# Autodesk Inventor assembly: main_frame
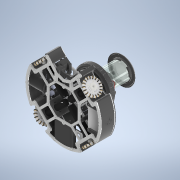
[picture p0: Inventor's stored thumbnail of the model, 180x180]
Saved by Autodesk Inventor 2020 (Build 240168000, 168)
## iProperties
Created: 2024-04-30
Part Number: main_frame
Document SubType Name: Assembly
Designer: 4s
Author: 4s
## Documents named in this file (25)
- C:\Users\4s\Documents\Inventor models\Asterisk\robot_v2\main_frame.iam
- C:\Users\4s\Documents\Inventor models\Asterisk\robot_v2\bottom_plate_v2.ipt
- C:\Users\4s\Documents\Inventor models\Asterisk\robot_v2\maxon mounts\back_mount.ipt
- C:\Users\4s\Documents\Inventor models\Asterisk\robot_v2\maxon mounts\left_mount.ipt
- C:\Users\4s\Documents\Inventor models\Asterisk\robot_v2\maxon mounts\right_mount.ipt
- C:\Users\4s\Documents\Inventor models\Asterisk\robot_v2\maxon motor\maxon motor.iam
- C:\Users\4s\Documents\Inventor models\Asterisk\robot_v2\maxon mounts\inner_mount.ipt
- C:\Users\4s\Documents\Inventor models\Asterisk\robot_v2\side_prot_cap.ipt
- C:\Users\4s\Documents\Inventor models\Asterisk\robot_v2\side_prot_stab_60.ipt
- C:\Users\4s\Documents\Inventor models\Asterisk\robot_v2\Bat_mount\bat_bed003_clear.ipt
- C:\Users\4s\Documents\Inventor models\Asterisk\robot_v2\a1401220.ipt
- C:\Users\4s\Documents\Inventor models\Asterisk\robot_v2\kicker\kicker_base_v7.ipt
- C:\Users\4s\Documents\Inventor models\Asterisk\robot_v2\upper_plate_v2.ipt
- C:\Users\4s\Documents\Inventor models\Asterisk\robot_v2\GTF Robots 50mm Wheel.ipt
- C:\Users\4s\Documents\Inventor models\Asterisk\robot_v2\board_support.ipt
- C:\Users\4s\Documents\Inventor models\Asterisk\robot_v2\pcb_main_board\motherboard.ipt
- C:\Users\4s\Documents\Inventor models\Asterisk\robot_v2\upper_mount\tsop_mount_v5.ipt
- C:\Users\4s\Documents\Inventor models\Asterisk\robot_v2\pcb_tsop_board\asterisk_tsop_board.ipt
- C:\Users\4s\Documents\Inventor models\Asterisk\robot_v2\upper_mount\tsop_imu_v1.ipt
- C:\Users\4s\Documents\Inventor models\Asterisk\9Dof Razor IMU.ipt
- C:\Users\4s\Documents\Inventor models\Asterisk\robot_v2\upper_mount\optic_mount_v3.ipt
- C:\Users\4s\Documents\Inventor models\Asterisk\robot_v2\openmv\openmv_h7.ipt
- C:\Users\4s\Documents\Inventor models\Asterisk\robot_v2\tube_50.ipt
- C:\Users\4s\Documents\Inventor models\Asterisk\robot_v2\mirror_50.ipt
- C:\Users\4s\Documents\Inventor models\Asterisk\robot_v2\upper_mount\mirror_lock_v4.ipt
## Components (34 placed, 24 different names)
1. bottom_plate_v2:1 — Совмещение:1, Совмещение:2, Совмещение:3, Совмещение:4, Совмещение:5, Совмещение:6, Совмещение:7, Совмещение:8, Совмещение:9, Совмещение:10, Совмещение:11, Совмещение:12, Совмещение:22, Совмещение:24, Совмещение:26, Совмещение:28, Совмещение:41, Совмещение:42, Совмещение:43, Совмещение:44, Совмещение:45, Совмещение:46, Совмещение:47, Совмещение:48, Совмещение:49, Совмещение:52, Совмещение:53, Совмещение:54, Совмещение:55
2. back_mount:1 — Совмещение:7, Совмещение:8, Совмещение:9, Совмещение:32, Совмещение:34, Совмещение:58
3. back_mount:2 — Совмещение:10, Совмещение:11, Совмещение:12, Совмещение:29, Совмещение:33, Совмещение:60
4. left_mount:1 — Совмещение:4, Совмещение:5, Совмещение:6, Совмещение:31, Совмещение:35, Совмещение:64
5. right_mount:1 — Совмещение:1, Совмещение:2, Совмещение:3, Совмещение:30, Совмещение:36, Совмещение:62
6. inner_mount:1 — Совмещение:22, Совмещение:38
7. inner_mount:2 — Совмещение:24, Совмещение:39
8. inner_mount:3 — Совмещение:26, Совмещение:40
9. inner_mount:4 — Совмещение:28, Совмещение:37
10. maxon motor:1 [sub-assembly] — Совмещение:30, Совмещение:36, Совмещение:38, Совмещение:61
11. maxon motor:2 [sub-assembly] — Совмещение:31, Совмещение:35, Совмещение:39, Совмещение:63
12. maxon motor:3 [sub-assembly] — Совмещение:32, Совмещение:34, Совмещение:40, Совмещение:57
13. maxon motor:4 [sub-assembly] — Совмещение:29, Совмещение:33, Совмещение:37, Совмещение:59
14. side_prot_cap:1 — Совмещение:41, Совмещение:42, Совмещение:43
15. side_prot_stab_60:1 — Совмещение:44, Совмещение:45, Совмещение:46, Совмещение:50, Совмещение:51
16. bat_bed003_clear:1 — Совмещение:47, Совмещение:48, Совмещение:49
17. a1401220:1 — Совмещение:50, Угол:1, Совмещение:51
18. kicker_base_v7:1 — Совмещение:52, Совмещение:53, Совмещение:54
19. upper_plate_v2:1 — Совмещение:55, Совмещение:56, Заподлицо:1, Совмещение:65, Совмещение:66, Совмещение:67, Совмещение:71, Совмещение:72, Совмещение:73
20. GTF Robots 50mm Wheel:1 — Совмещение:57, Совмещение:58
21. GTF Robots 50mm Wheel:2 — Совмещение:59, Совмещение:60
22. GTF Robots 50mm Wheel:3 — Совмещение:61, Совмещение:62
23. GTF Robots 50mm Wheel:4 — Совмещение:63, Совмещение:64
24. board_support:1 — Совмещение:65, Совмещение:66, Совмещение:67, Совмещение:68, Совмещение:69, Совмещение:70
25. motherboard:1 — Совмещение:68, Совмещение:69, Совмещение:70
26. tsop_mount_v5:1 — Совмещение:71, Совмещение:72, Совмещение:73, Совмещение:74, Совмещение:75, Совмещение:76, Совмещение:77
27. asterisk_tsop_board:1 — Совмещение:74, Совмещение:75, Угол:2, Угол:3
28. tsop_imu_v1:1 — Совмещение:76, Совмещение:77, Совмещение:79, Совмещение:80, Совмещение:81, Угол:5, Совмещение:82
29. 9Dof Razor IMU:1 — Совмещение:78, Совмещение:79, Угол:4
30. optic_mount_v3:1 — Совмещение:80, Совмещение:81, Совмещение:82, Совмещение:83, Совмещение:84, Угол:6, Совмещение:85, Совмещение:86
31. openmv_h7:1 — Совмещение:83, Совмещение:84, Угол:6
32. tube_50:1 — Совмещение:85, Совмещение:86, Совмещение:87, Совмещение:88, Совмещение:89, Угол:7
33. mirror_50:1 — Совмещение:87, Совмещение:88, Совмещение:90
34. mirror_lock_v4:1 — Совмещение:89, Совмещение:90
## Relationships (86: Mate 78, Angle 7, Flush 1)
- Совмещение:1 [Mate]: bottom_plate_v2:1 ↔ right_mount:1
- Совмещение:2 [Mate]: bottom_plate_v2:1 ↔ right_mount:1
- Совмещение:3 [Mate]: bottom_plate_v2:1 ↔ right_mount:1
- Совмещение:4 [Mate]: bottom_plate_v2:1 ↔ left_mount:1
- Совмещение:5 [Mate]: bottom_plate_v2:1 ↔ left_mount:1
- Совмещение:6 [Mate]: bottom_plate_v2:1 ↔ left_mount:1
- Совмещение:7 [Mate]: bottom_plate_v2:1 ↔ back_mount:1
- Совмещение:8 [Mate]: bottom_plate_v2:1 ↔ back_mount:1
- Совмещение:9 [Mate]: bottom_plate_v2:1 ↔ back_mount:1
- Совмещение:10 [Mate]: bottom_plate_v2:1 ↔ back_mount:2
- Совмещение:11 [Mate]: bottom_plate_v2:1 ↔ back_mount:2
- Совмещение:12 [Mate]: bottom_plate_v2:1 ↔ back_mount:2
- Совмещение:22 [Mate]: bottom_plate_v2:1 ↔ inner_mount:1
- Совмещение:24 [Mate]: bottom_plate_v2:1 ↔ inner_mount:2
- Совмещение:26 [Mate]: bottom_plate_v2:1 ↔ inner_mount:3
- Совмещение:28 [Mate]: bottom_plate_v2:1 ↔ inner_mount:4
- Совмещение:29 [Mate]: back_mount:2 ↔ maxon motor:4
- Совмещение:30 [Mate]: right_mount:1 ↔ maxon motor:1
- Совмещение:31 [Mate]: left_mount:1 ↔ maxon motor:2
- Совмещение:32 [Mate]: back_mount:1 ↔ maxon motor:3
- Совмещение:33 [Mate]: back_mount:2 ↔ maxon motor:4
- Совмещение:34 [Mate]: back_mount:1 ↔ maxon motor:3
- Совмещение:35 [Mate]: left_mount:1 ↔ maxon motor:2
- Совмещение:36 [Mate]: right_mount:1 ↔ maxon motor:1
- Совмещение:37 [Mate]: inner_mount:4 ↔ maxon motor:4
- Совмещение:38 [Mate]: inner_mount:1 ↔ maxon motor:1
- Совмещение:39 [Mate]: inner_mount:2 ↔ maxon motor:2
- Совмещение:40 [Mate]: inner_mount:3 ↔ maxon motor:3
- Совмещение:41 [Mate]: bottom_plate_v2:1 ↔ side_prot_cap:1
- Совмещение:42 [Mate]: bottom_plate_v2:1 ↔ side_prot_cap:1
- Совмещение:43 [Mate]: bottom_plate_v2:1 ↔ side_prot_cap:1
- Совмещение:44 [Mate]: bottom_plate_v2:1 ↔ side_prot_stab_60:1
- Совмещение:45 [Mate]: bottom_plate_v2:1 ↔ side_prot_stab_60:1
- Совмещение:46 [Mate]: bottom_plate_v2:1 ↔ side_prot_stab_60:1
- Совмещение:47 [Mate]: bottom_plate_v2:1 ↔ bat_bed003_clear:1
- Совмещение:48 [Mate]: bottom_plate_v2:1 ↔ bat_bed003_clear:1
- Совмещение:49 [Mate]: bottom_plate_v2:1 ↔ bat_bed003_clear:1
- Совмещение:50 [Mate]: side_prot_stab_60:1 ↔ a1401220:1
- Угол:1 [Angle] (0 deg): a1401220:1
- Совмещение:51 [Mate]: side_prot_stab_60:1 ↔ a1401220:1
- Совмещение:52 [Mate]: bottom_plate_v2:1 ↔ kicker_base_v7:1
- Совмещение:53 [Mate]: bottom_plate_v2:1 ↔ kicker_base_v7:1
- Совмещение:54 [Mate]: bottom_plate_v2:1 ↔ kicker_base_v7:1
- Совмещение:55 [Mate] (35 mm): bottom_plate_v2:1 ↔ upper_plate_v2:1
- Совмещение:56 [Mate]: upper_plate_v2:1
- Заподлицо:1 [Flush]: upper_plate_v2:1
- Совмещение:57 [Mate]: maxon motor:3 ↔ GTF Robots 50mm Wheel:1
- Совмещение:58 [Mate] (1.5 mm): back_mount:1 ↔ GTF Robots 50mm Wheel:1
- Совмещение:59 [Mate]: maxon motor:4 ↔ GTF Robots 50mm Wheel:2
- Совмещение:60 [Mate] (1.5 mm): back_mount:2 ↔ GTF Robots 50mm Wheel:2
- Совмещение:61 [Mate]: maxon motor:1 ↔ GTF Robots 50mm Wheel:3
- Совмещение:62 [Mate] (1.5 mm): right_mount:1 ↔ GTF Robots 50mm Wheel:3
- Совмещение:63 [Mate]: maxon motor:2 ↔ GTF Robots 50mm Wheel:4
- Совмещение:64 [Mate] (1.5 mm): left_mount:1 ↔ GTF Robots 50mm Wheel:4
- Совмещение:65 [Mate]: upper_plate_v2:1 ↔ board_support:1
- Совмещение:66 [Mate]: upper_plate_v2:1 ↔ board_support:1
- Совмещение:67 [Mate]: upper_plate_v2:1 ↔ board_support:1
- Совмещение:68 [Mate]: board_support:1 ↔ motherboard:1
- Совмещение:69 [Mate]: board_support:1 ↔ motherboard:1
- Совмещение:70 [Mate]: board_support:1 ↔ motherboard:1
- Совмещение:71 [Mate]: upper_plate_v2:1 ↔ tsop_mount_v5:1
- Совмещение:72 [Mate]: upper_plate_v2:1 ↔ tsop_mount_v5:1
- Совмещение:73 [Mate]: upper_plate_v2:1 ↔ tsop_mount_v5:1
- Совмещение:74 [Mate]: tsop_mount_v5:1 ↔ asterisk_tsop_board:1
- Совмещение:75 [Mate]: tsop_mount_v5:1 ↔ asterisk_tsop_board:1
- Угол:2 [Angle] (0 deg): asterisk_tsop_board:1
- Совмещение:76 [Mate]: tsop_mount_v5:1 ↔ tsop_imu_v1:1
- Совмещение:77 [Mate]: tsop_mount_v5:1 ↔ tsop_imu_v1:1
- Угол:3 [Angle] (0 deg): asterisk_tsop_board:1
- Совмещение:78 [Mate]: 9Dof Razor IMU:1
- Совмещение:79 [Mate]: tsop_imu_v1:1 ↔ 9Dof Razor IMU:1
- Угол:4 [Angle] (0 deg): 9Dof Razor IMU:1
- Совмещение:80 [Mate]: tsop_imu_v1:1 ↔ optic_mount_v3:1
- Совмещение:81 [Mate]: tsop_imu_v1:1 ↔ optic_mount_v3:1
- Угол:5 [Angle] (0 deg): tsop_imu_v1:1
- Совмещение:82 [Mate]: tsop_imu_v1:1 ↔ optic_mount_v3:1
- Совмещение:83 [Mate]: optic_mount_v3:1 ↔ openmv_h7:1
- Совмещение:84 [Mate]: optic_mount_v3:1 ↔ openmv_h7:1
- Угол:6 [Angle] (0 deg): optic_mount_v3:1 ↔ openmv_h7:1
- Совмещение:85 [Mate]: optic_mount_v3:1 ↔ tube_50:1
- Совмещение:86 [Mate]: optic_mount_v3:1 ↔ tube_50:1
- Совмещение:87 [Mate]: tube_50:1 ↔ mirror_50:1
- Совмещение:88 [Mate]: tube_50:1 ↔ mirror_50:1
- Совмещение:89 [Mate]: tube_50:1 ↔ mirror_lock_v4:1
- Совмещение:90 [Mate]: mirror_50:1 ↔ mirror_lock_v4:1
- Угол:7 [Angle] (0 deg): tube_50:1
